# Autodesk Inventor assembly: EvelShortFrontFrame
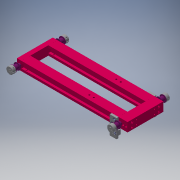
[picture p0: Inventor's stored thumbnail of the model, 180x180]
Saved by Autodesk Inventor 2019 (Build 230136000, 136)
## iProperties
Created: 2019-09-29
Part Number: EvelShortFrontFrame
Document SubType Name: Weldment
Designer: james
Weld Material: Welded Aluminum-6061
Author: james
## Documents named in this file (4)
- F:\JimsDesign\Jims2020FTC\EvelShortFrontFrame.iam
- F:\JimsDesign\Jims2020FTC\SliderRight.iam
- F:\JimsDesign\Jims2020FTC\FullElevatorShart.iam
- F:\JimsDesign\Jims2020FTC\ShortElevatorFrame.iam
## Components (5 placed, 3 different names)
1. ShortElevatorFrame:1 [sub-assembly] — Mate:1, Mate:11, Mate:12, Mate:19, Mate:21, Mate:22, Mate:23, Mate:24
2. SliderRight:1 [sub-assembly] — Mate:24, Flush:1, Flush:2
3. FullElevatorShart:1 [sub-assembly] — Mate:12, Mate:19
4. FullElevatorShart:2 [sub-assembly] — Mate:1, Mate:11
5. SliderRight:2 [sub-assembly] — Mate:21, Mate:22, Mate:23, Flush:1, Flush:2
## Relationships (10: Mate 8, Flush 2)
- Mate:1: ShortElevatorFrame:1 ↔ FullElevatorShart:2
- Mate:11: ShortElevatorFrame:1 ↔ FullElevatorShart:2
- Mate:12: ShortElevatorFrame:1 ↔ FullElevatorShart:1
- Mate:19: ShortElevatorFrame:1 ↔ FullElevatorShart:1
- Mate:21: ShortElevatorFrame:1 ↔ SliderRight:2
- Mate:22: ShortElevatorFrame:1 ↔ SliderRight:2
- Mate:23: ShortElevatorFrame:1 ↔ SliderRight:2
- Mate:24: ShortElevatorFrame:1 ↔ SliderRight:1
- Flush:1: SliderRight:1 ↔ SliderRight:2
- Flush:2: SliderRight:1 ↔ SliderRight:2
